# Autodesk Inventor assembly: Base with Cover
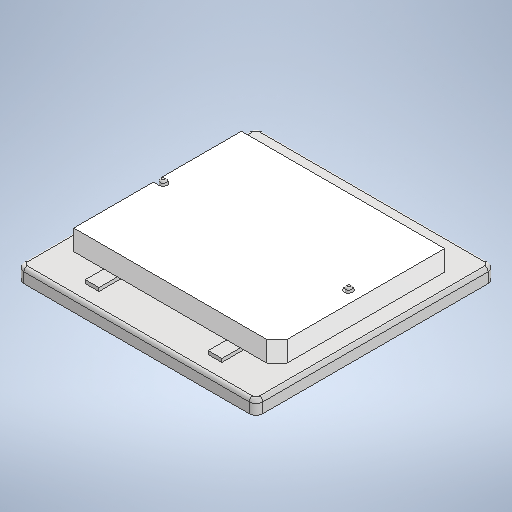
[picture p0: Inventor's stored thumbnail of the model, 512x512]
Saved by Autodesk Inventor 2025 (Build 290162000, 162)
## iProperties
Created: 2025-02-28
Part Number: Base with Cover
Document SubType Name: Assembly
Designer: Caleb Fangmeier
Author: Caleb Fangmeier
## Documents named in this file (3)
- C:\Users\cfang\Desktop\nebraska-silicon-lab\Hardware\ETL\Module Assembly\Digital Module Cover V3\Base with Cover.iam
- C:\Users\cfang\Desktop\nebraska-silicon-lab\Hardware\ETL\Module Assembly\Digital Module Cover V3\Digital Module Cover V3.ipt
- C:\Users\cfang\Desktop\nebraska-silicon-lab\Hardware\ETL\Module Assembly\Digital Module Cover V3\Installation Base.ipt
## Components (2 placed, 2 different names)
1. Digital Module Cover V3:1 — Mate:1, Angle:1
2. Installation Base:1 — Mate:1, Angle:1
## Relationships (2: Mate 1, Angle 1)
- Mate:1: Digital Module Cover V3:1 ↔ Installation Base:1
- Angle:1 (0 deg): Digital Module Cover V3:1 ↔ Installation Base:1
